# Autodesk Inventor assembly: Rope Climber
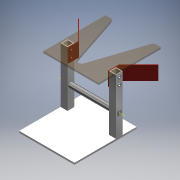
[picture p0: Inventor's stored thumbnail of the model, 180x180]
Saved by Autodesk Inventor 2018.2 (Build 222227000, 227)
## iProperties
Created: 2017-03-26
Part Number: Rope Climber
Document SubType Name: Assembly
Designer: steele
Mass: 1594.06 g
Surface Area: 2896.68 cm^2
Volume: 625.96 cm^3
Density: 2.54658 g/cm^3
Author: steele
## Documents named in this file (8)
- D:\snobotics\CAD-Development\robSteele\2018-FRC\RobotLiftMechanism\Rope Climber.iam
- D:\snobotics\CAD-Development\robSteele\SnoBotics2017\Rope Climber\basePlate.ipt
- D:\snobotics\CAD-Development\robSteele\SnoBotics2017\Rope Climber\Post.ipt
- D:\snobotics\CAD-Development\robSteele\SnoBotics2017\Rope Climber\Guide.ipt
- D:\snobotics\CAD-Development\robSteele\SnoBotics2017\Rope Climber\Rope Climber\Design Accelerator\Bolted Connection1.iam
- D:\snobotics\CAD-Development\robSteele\SnoBotics2017\Rope Climber\Rope Climber\Design Accelerator\Bolted Connection2.iam
- D:\snobotics\CAD-Development\robSteele\SnoBotics2017\Rope Climber\lexanRopeGuide.ipt
- D:\snobotics\CAD-Development\robSteele\SnoBotics2017\Rope Climber\ropeClimberAxel.ipt
## Components (9 placed, 6 different names)
1. basePlate:1 — Mate:1, Flush:1, Flush:2, Mate:2, Flush:3, Flush:4, Mate:12
2. Post:1 — Mate:1, Flush:1, Flush:2, Mate:3, Flush:5, Flush:6, Mate:9, Flush:9, Flush:10, Flush:12
3. Post:2 — Mate:2, Flush:3, Flush:4, Mate:4, Flush:7, Flush:8, Mate:11
4. Guide:1 — Mate:3, Flush:5, Flush:6, Mate:5, Mate:6
5. Guide:2 — Mate:4, Flush:7, Flush:8, Mate:7, Mate:8
6. Bolted Connection:1 [sub-assembly] — Mate:5, Mate:6
7. Bolted Connection:2 [sub-assembly] — Mate:7, Mate:8
8. lexanRopeGuide:1 — Mate:9, Flush:9, Flush:10
9. ropeClimberAxel:1 — Mate:10, Mate:11, Mate:12
## Relationships (23: Mate 12, Flush 11)
- Mate:1: basePlate:1 ↔ Post:1
- Flush:1: basePlate:1 ↔ Post:1
- Flush:2 (-152.4 mm): basePlate:1 ↔ Post:1
- Mate:2: basePlate:1 ↔ Post:2
- Flush:3: basePlate:1 ↔ Post:2
- Flush:4 (-152.4 mm): basePlate:1 ↔ Post:2
- Mate:3: Post:1 ↔ Guide:1
- Flush:5: Post:1 ↔ Guide:1
- Flush:6: Post:1 ↔ Guide:1
- Mate:4: Post:2 ↔ Guide:2
- Flush:7: Post:2 ↔ Guide:2
- Flush:8: Post:2 ↔ Guide:2
- Mate:5: Guide:1 ↔ Bolted Connection:1
- Mate:6: Guide:1 ↔ Bolted Connection:1
- Mate:7: Guide:2 ↔ Bolted Connection:2
- Mate:8: Guide:2 ↔ Bolted Connection:2
- Mate:9: Post:1 ↔ lexanRopeGuide:1
- Flush:9 (63.5 mm): Post:1 ↔ lexanRopeGuide:1
- Flush:10: Post:1 ↔ lexanRopeGuide:1
- Flush:12 (76.2 mm): Post:1
- Mate:10: ropeClimberAxel:1
- Mate:11 (-12.7 mm): Post:2 ↔ ropeClimberAxel:1
- Mate:12 (76.2 mm): basePlate:1 ↔ ropeClimberAxel:1
